# Autodesk Inventor assembly: Nose assembly
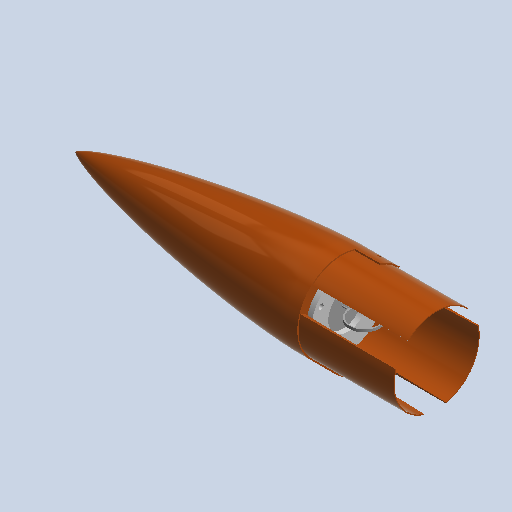
[picture p0: Inventor's stored thumbnail of the model, 512x512]
Saved by Autodesk Inventor 2024 (Build 280153000, 153)
## iProperties
Part Number: Nose assembly
Document SubType Name: Assembly
Designer: Jamie
Author: Jamie
## Documents named in this file (4)
- C:\Users\auror\Documents\TU Delft\DARE\Git\Scrambler-2-CAD\Autodesk\Nose assembly.iam
- C:\Users\auror\Documents\TU Delft\DARE\Git\Scrambler-2-CAD\Autodesk\smoke_grenade.ipt
- C:\Users\auror\Documents\TU Delft\DARE\Git\Scrambler-2-CAD\Autodesk\Nosecone.ipt
- C:\Users\auror\Documents\TU Delft\DARE\Git\Scrambler-2-CAD\Autodesk\grenade_retention_ring.ipt
## Components (3 placed, 3 different names)
1. smoke_grenade:1 — Mate:1, Mate:2, Rotational:1
2. Nosecone:1 — Mate:1, Mate:2
3. grenade_retention_ring:1 — Rotational:1
## Relationships (3: Mate 2, RevoluteJoint 1)
- Mate:1: smoke_grenade:1 ↔ Nosecone:1
- Mate:2: smoke_grenade:1 ↔ Nosecone:1
- Rotational:1 [RevoluteJoint] (5 mm): smoke_grenade:1 ↔ grenade_retention_ring:1
